# Autodesk Inventor assembly: Height Adjustment Frame
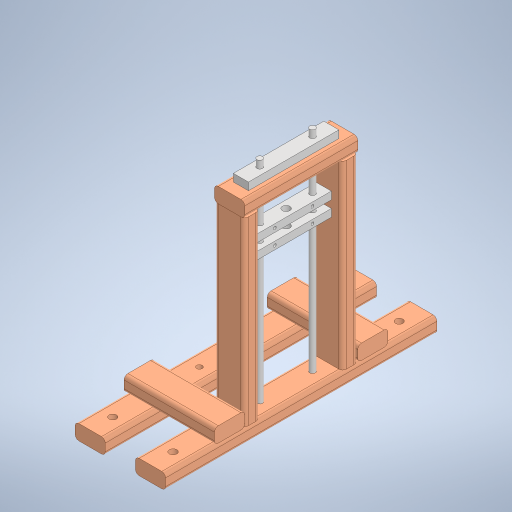
[picture p0: Inventor's stored thumbnail of the model, 512x512]
Saved by Autodesk Inventor 2024 (Build 280153000, 153)
## iProperties
Created: 2024-03-20
Part Number: Height Adjustment Frame
Document SubType Name: Assembly
Designer: Liz
Author: Liz
## Documents named in this file (8)
- C:\Users\anyangoe\Desktop\WholeRobot\Height Adjustment Frame.iam
- C:\Users\anyangoe\Desktop\WholeRobot\Metal Bar-1.ipt
- C:\Users\anyangoe\Desktop\WholeRobot\Metal Bar-2.ipt
- C:\Users\anyangoe\Desktop\WholeRobot\Metal Rod.ipt
- C:\Users\anyangoe\Desktop\WholeRobot\Wood-1.ipt
- C:\Users\anyangoe\Desktop\WholeRobot\Wood-2.ipt
- C:\Users\anyangoe\Desktop\WholeRobot\Wood-3.ipt
- C:\Users\anyangoe\Desktop\WholeRobot\Wood-4.ipt
## Components (12 placed, 7 different names)
1. Metal Bar-1:1 — Mate:8, Mate:9, Mate:10
2. Metal Bar-2:1 — Mate:11, Mate:12, Mate:20, Mate:21
3. Metal Rod:1 — Mate:2, Flush:2, Mate:4, Mate:9, Mate:12, Mate:14
4. Wood-1:1 — Mate:3, Mate:4, Flush:4, Mate:6, Mate:7, Flush:7, Mate:10, Mate:21
5. Wood-2:1 — Mate:5, Flush:4, Mate:6, Flush:5, Mate:17
6. Wood-3:1 — Mate:16, Flush:9, Mate:18, Mate:19, Flush:11
7. Wood-4:1 — Mate:19, Flush:10, Flush:11
8. Metal Rod:2 — Mate:1, Flush:1, Mate:3, Mate:8, Mate:11, Mate:13
9. Wood-2:2 — Flush:6, Mate:7, Flush:7, Mate:18
10. Wood-4:2 — Mate:1, Mate:2, Flush:1, Flush:2, Mate:5, Flush:5, Flush:6, Mate:15, Mate:16, Flush:8, Flush:9, Flush:10
11. Metal Bar-2:2 — Mate:13, Mate:14, Mate:20
12. Wood-3:2 — Mate:15, Flush:8, Mate:17
## Relationships (31: Mate 21, Flush 10)
- Mate:1: Metal Rod:2 ↔ Wood-4:2
- Mate:2: Metal Rod:1 ↔ Wood-4:2
- Flush:1: Metal Rod:2 ↔ Wood-4:2
- Flush:2: Metal Rod:1 ↔ Wood-4:2
- Mate:3: Wood-1:1 ↔ Metal Rod:2
- Mate:4: Metal Rod:1 ↔ Wood-1:1
- Mate:5: Wood-2:1 ↔ Wood-4:2
- Flush:4: Wood-1:1 ↔ Wood-2:1
- Mate:6: Wood-1:1 ↔ Wood-2:1
- Flush:5: Wood-2:1 ↔ Wood-4:2
- Flush:6: Wood-2:2 ↔ Wood-4:2
- Mate:7: Wood-1:1 ↔ Wood-2:2
- Flush:7: Wood-1:1 ↔ Wood-2:2
- Mate:8: Metal Bar-1:1 ↔ Metal Rod:2
- Mate:9: Metal Bar-1:1 ↔ Metal Rod:1
- Mate:10: Metal Bar-1:1 ↔ Wood-1:1
- Mate:11: Metal Bar-2:1 ↔ Metal Rod:2
- Mate:12: Metal Bar-2:1 ↔ Metal Rod:1
- Mate:13: Metal Rod:2 ↔ Metal Bar-2:2
- Mate:14: Metal Rod:1 ↔ Metal Bar-2:2
- Mate:15: Wood-4:2 ↔ Wood-3:2
- Mate:16: Wood-3:1 ↔ Wood-4:2
- Flush:8: Wood-4:2 ↔ Wood-3:2
- Flush:9: Wood-3:1 ↔ Wood-4:2
- Mate:17: Wood-2:1 ↔ Wood-3:2
- Mate:18: Wood-3:1 ↔ Wood-2:2
- Mate:19: Wood-3:1 ↔ Wood-4:1
- Flush:10: Wood-4:1 ↔ Wood-4:2
- Flush:11: Wood-3:1 ↔ Wood-4:1
- Mate:20 (-76.2 mm): Metal Bar-2:1 ↔ Metal Bar-2:2
- Mate:21 (457.2 mm): Metal Bar-2:1 ↔ Wood-1:1
